# Autodesk Inventor assembly: protoswitchboard
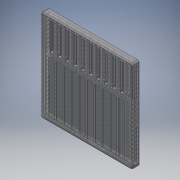
[picture p0: Inventor's stored thumbnail of the model, 180x180]
Saved by Autodesk Inventor 2017 (Build 210142000, 142)
## iProperties
Created: 2017-08-24
Part Number: protoswitchboard
Document SubType Name: Assembly
Designer: erwin
Author: erwin
## Documents named in this file (3)
- D:\GitHub\ProtoSwitchBoard\4\protoswitchboard.iam
- D:\GitHub\ProtoSwitchBoard\3\cover.ipt
- D:\GitHub\ProtoSwitchBoard\3\bottom.ipt
## Components (2 placed, 2 different names)
1. cover:1 — Flush:1, Flush:2, Flush:3, Flush:4
2. bottom:1 — Flush:1, Flush:2, Flush:3, Flush:4
## Relationships (4: Flush 4)
- Flush:1: cover:1 ↔ bottom:1
- Flush:2: cover:1 ↔ bottom:1
- Flush:3 (0.3 mm): cover:1 ↔ bottom:1
- Flush:4 (-3.75 mm): cover:1 ↔ bottom:1
